# Autodesk Inventor assembly: Assembly1
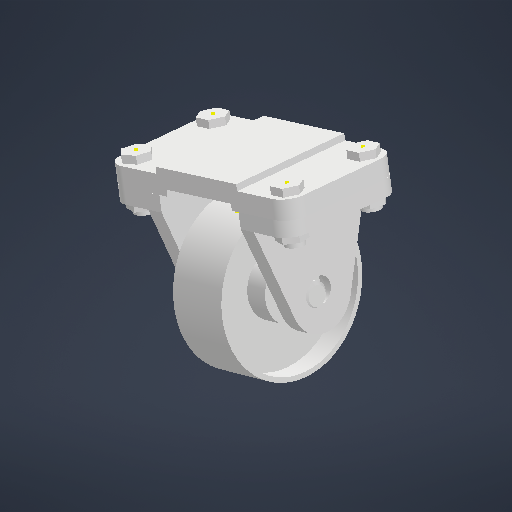
[picture p0: Inventor's stored thumbnail of the model, 512x512]
Saved by Autodesk Inventor 2026 (Build 300175000, 175)
## iProperties
Created: 2025-05-07
Part Number: Assembly1
Document SubType Name: Assembly
Designer: Ritul Kumari
Author: Ritul Kumari
## Documents named in this file (7)
- C:\Users\Ritul Kumari\Documents\Inventor\inventor P1\Assembly1.iam
- C:\Users\Ritul Kumari\Documents\Inventor\inventor P1\Part4.ipt
- C:\Users\Ritul Kumari\Documents\Inventor\inventor P1\Wheel.ipt
- C:\Users\Ritul Kumari\Documents\Inventor\inventor P1\axle support.ipt
- C:\Users\Ritul Kumari\Documents\Inventor\inventor P1\axle.ipt
- C:\Users\Ritul Kumari\Documents\Inventor\inventor P1\nut2.ipt
- C:\Users\Ritul Kumari\Documents\Inventor\inventor P1\Bolt.ipt
## Components (13 placed, 6 different names)
1. Part4:1 — Insert:1, Insert:2, Insert:11, Insert:12, Rotational:1, Rotational:2, Rotational:3, Rotational:4, Rotational:5
2. Wheel:1 — Insert:10
3. axle support:1 — Insert:2, Insert:12, Rotational:1, Rotational:2, Insert:13, Insert:14
4. axle support:2 — Insert:1, Insert:15, Insert:16
5. axle:1 — Insert:10
6. nut2:1 — Rotational:3
7. nut2:2 — Insert:11
8. nut2:3 — Rotational:5
9. nut2:4 — Rotational:4
10. Bolt:1 — Insert:13
11. Bolt:2 — Insert:16
12. Bolt:3 — Insert:14
13. Bolt:4 — Insert:15
## Relationships (14: Insert 9, RevoluteJoint 5)
- Insert:1: Part4:1 ↔ axle support:2
- Insert:2: Part4:1 ↔ axle support:1
- Insert:10: Wheel:1 ↔ axle:1
- Insert:11: Part4:1 ↔ nut2:2
- Insert:12: Part4:1 ↔ axle support:1
- Rotational:1 [RevoluteJoint]: Part4:1 ↔ axle support:1
- Rotational:2 [RevoluteJoint]: Part4:1 ↔ axle support:1
- Rotational:3 [RevoluteJoint]: Part4:1 ↔ nut2:1
- Rotational:4 [RevoluteJoint]: Part4:1 ↔ nut2:4
- Rotational:5 [RevoluteJoint]: Part4:1 ↔ nut2:3
- Insert:13: axle support:1 ↔ Bolt:1
- Insert:14: axle support:1 ↔ Bolt:3
- Insert:15: axle support:2 ↔ Bolt:4
- Insert:16: axle support:2 ↔ Bolt:2
